# Autodesk Inventor assembly: Structure
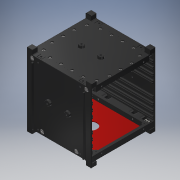
[picture p0: Inventor's stored thumbnail of the model, 180x180]
Saved by Autodesk Inventor 2018 (Build 220112000, 112)
## iProperties
Created: 2018-07-04
Part Number: Structure
Document SubType Name: Assembly
Designer: Bradley
Mass: 378.313 g
Surface Area: 1634.79 cm^2
Volume: 135.905 cm^3
Density: 2.78366 g/cm^3
Author: Bradley
## Documents named in this file (14)
- D:\Users\Bradley\Documents\CougsInSpace\CougSat1-Hardware\CougSat1-Structure\CADModel\Native\Structure.iam
- D:\Users\Bradley\Documents\CougsInSpace\CougSat1-Hardware\CougSat1-Structure\CADModel\Native\Structure_Y.ipt
- D:\Users\Bradley\Documents\CougsInSpace\CougSat1-Hardware\CougSat1-Structure\CADModel\Native\Structure_+Z.ipt
- D:\Users\Bradley\Documents\CougsInSpace\CougSat1-Hardware\CougSat1-Structure\CADModel\Native\Structure_-Z.ipt
- D:\Users\Bradley\Documents\CougsInSpace\CougSat1-Hardware\CougSat1-Structure\CADModel\Native\Structure_+X.ipt
- D:\Users\Bradley\Documents\CougsInSpace\CougSat1-Hardware\CougSat1-Structure\CADModel\Native\Structure_-X.ipt
- D:\Users\Bradley\Documents\CougsInSpace\Resources\ComponentModels\Hardware\Spring_Separation.ipt
- D:\Users\Bradley\Documents\CougsInSpace\Resources\ComponentModels\Electronics\Switch_Micro-L.iam
- D:\Users\Bradley\Documents\CougsInSpace\Resources\ComponentModels\Hardware\Pin_Headed-2x6mm.ipt
- D:\Users\Bradley\Documents\CougsInSpace\Resources\ComponentModels\Fasteners\Bolt_M1.6x0.35_5mm_SH.ipt
- D:\Users\Bradley\Documents\CougsInSpace\Resources\ComponentModels\Fasteners\Bolt_M2x0.4_8mm_SH.ipt
- D:\Users\Bradley\Documents\CougsInSpace\CougSat1-Hardware\CougSat1-Structure\CADModel\Native\Structure_-ZCover.ipt
- D:\Users\Bradley\Documents\CougsInSpace\Resources\ComponentModels\Fasteners\Bolt_M2x0.4_4mm_SH.ipt
- D:\Users\Bradley\Documents\CougsInSpace\Resources\ComponentModels\Fasteners\Bolt_M3x0.35_10mm_LSH.ipt
## Components (47 placed, 13 different names)
1. Structure_+X:1 — Mate:1, Flush:6, Flush:7, Insert:16, Insert:19
2. Structure_Y:1 — Flush:3, Flush:4, Insert:5, Insert:6, Insert:7, Insert:8, Insert:11, Insert:12, Insert:13, Insert:22, Insert:30, Insert:31, Insert:32
3. Structure_+Z:1 — Insert:9, Insert:10, Insert:11, Insert:12, Flush:5, Mate:1, Insert:16, Insert:17, Insert:18, Insert:33, Insert:34, Insert:35, Insert:36, Insert:37, Insert:38, Insert:39, Insert:40, Insert:41, Insert:42, Insert:43, Insert:44, Insert:45, Insert:46, Insert:47, Insert:48, Insert:49, Insert:50
4. Structure_-X:1 — Insert:17, Insert:18, Insert:20
5. Structure_Y:2 — Mate:2, Insert:1, Insert:2, Insert:3, Insert:4, Insert:9, Insert:10, Insert:14, Insert:15, Insert:21, Insert:25, Insert:26, Insert:27
6. Structure_-Z:1 — Insert:13, Insert:14, Insert:15, Insert:19, Insert:20, Insert:51, Insert:52
7. Structure_-ZCover:1 — Insert:51, Insert:52, Insert:53, Insert:54, Insert:55, Insert:56
8. Switch_Micro-L:1 [sub-assembly] — Insert:23, Insert:24, Insert:26, Insert:27, Tangent:1
9. Switch_Micro-L:2 [sub-assembly] — Insert:30, Insert:31
10. Bolt_M1.6x0.35_5mm_SH:1 — Insert:24
11. Bolt_M1.6x0.35_5mm_SH:2 — Insert:23
12. Bolt_M1.6x0.35_5mm_SH:3
13. Bolt_M1.6x0.35_5mm_SH:4
14. Bolt_M2x0.4_4mm_SH:1 — Insert:53
15. Bolt_M2x0.4_4mm_SH:2 — Insert:54
16. Bolt_M2x0.4_4mm_SH:3 — Insert:55
17. Bolt_M2x0.4_4mm_SH:4 — Insert:56
18. Bolt_M2x0.4_8mm_SH:1 — Insert:33
19. Bolt_M2x0.4_8mm_SH:2 — Insert:34
20. Bolt_M2x0.4_8mm_SH:3 — Insert:35
21. Bolt_M2x0.4_8mm_SH:4 — Insert:36
22. Bolt_M2x0.4_8mm_SH:5 — Insert:37
23. Bolt_M2x0.4_8mm_SH:6 — Insert:38
24. Bolt_M2x0.4_8mm_SH:7 — Insert:39
25. Bolt_M2x0.4_8mm_SH:8 — Insert:40
26. Bolt_M2x0.4_8mm_SH:9 — Insert:41
27. Bolt_M2x0.4_8mm_SH:10 — Insert:42
28. Bolt_M2x0.4_8mm_SH:11 — Insert:43
29. Bolt_M2x0.4_8mm_SH:12 — Insert:44
30. Bolt_M2x0.4_8mm_SH:13 — Insert:45
31. Bolt_M2x0.4_8mm_SH:14 — Insert:46
32. Bolt_M2x0.4_8mm_SH:15 — Insert:47
33. Bolt_M2x0.4_8mm_SH:16 — Insert:48
34. Bolt_M2x0.4_8mm_SH:17 — Insert:49
35. Bolt_M2x0.4_8mm_SH:18 — Insert:50
36. Bolt_M3x0.35_10mm_LSH:1 — Insert:1
37. Bolt_M3x0.35_10mm_LSH:2 — Insert:2
38. Bolt_M3x0.35_10mm_LSH:3 — Insert:3
39. Bolt_M3x0.35_10mm_LSH:4 — Insert:4
40. Bolt_M3x0.35_10mm_LSH:5 — Insert:5
41. Bolt_M3x0.35_10mm_LSH:6 — Insert:7
42. Bolt_M3x0.35_10mm_LSH:7 — Insert:6
43. Bolt_M3x0.35_10mm_LSH:8 — Insert:8
44. Pin_Headed-2x6mm:1 — Insert:25, Tangent:1
45. Pin_Headed-2x6mm:2 — Insert:32
46. Spring_Separation:1 — Insert:22
47. Spring_Separation:2 — Insert:21
## Relationships (66: Insert 56, Flush 6, Mate 2, Tangent 2)
- Mate:2: Structure_Y:2
- [Flush]: Structure_Y:2
- Flush:3: Structure_Y:1
- Flush:4: Structure_Y:1
- Insert:1: Structure_Y:2 ↔ Bolt_M3x0.35_10mm_LSH:1
- Insert:2: Structure_Y:2 ↔ Bolt_M3x0.35_10mm_LSH:2
- Insert:3: Structure_Y:2 ↔ Bolt_M3x0.35_10mm_LSH:3
- Insert:4: Structure_Y:2 ↔ Bolt_M3x0.35_10mm_LSH:4
- Insert:5: Structure_Y:1 ↔ Bolt_M3x0.35_10mm_LSH:5
- Insert:6: Structure_Y:1 ↔ Bolt_M3x0.35_10mm_LSH:7
- Insert:7: Structure_Y:1 ↔ Bolt_M3x0.35_10mm_LSH:6
- Insert:8: Structure_Y:1 ↔ Bolt_M3x0.35_10mm_LSH:8
- Insert:9: Structure_+Z:1 ↔ Structure_Y:2
- Insert:10: Structure_+Z:1 ↔ Structure_Y:2
- Insert:11: Structure_Y:1 ↔ Structure_+Z:1
- Insert:12: Structure_Y:1 ↔ Structure_+Z:1
- Flush:5: Structure_+Z:1
- Insert:13: Structure_Y:1 ↔ Structure_-Z:1
- Insert:14: Structure_Y:2 ↔ Structure_-Z:1
- Insert:15: Structure_Y:2 ↔ Structure_-Z:1
- Mate:1: Structure_+X:1 ↔ Structure_+Z:1
- Flush:6: Structure_+X:1
- Flush:7: Structure_+X:1
- Insert:16: Structure_+X:1 ↔ Structure_+Z:1
- Insert:17: Structure_+Z:1 ↔ Structure_-X:1
- Insert:18: Structure_+Z:1 ↔ Structure_-X:1
- Insert:19: Structure_+X:1 ↔ Structure_-Z:1
- Insert:20: Structure_-X:1 ↔ Structure_-Z:1
- Insert:21: Structure_Y:2 ↔ Spring_Separation:2
- Insert:22: Structure_Y:1 ↔ Spring_Separation:1
- Insert:23: Switch_Micro-L:1 ↔ Bolt_M1.6x0.35_5mm_SH:2
- Insert:24: Switch_Micro-L:1 ↔ Bolt_M1.6x0.35_5mm_SH:1
- Insert:25: Structure_Y:2 ↔ Pin_Headed-2x6mm:1
- Insert:26: Structure_Y:2 ↔ Switch_Micro-L:1
- Insert:27: Structure_Y:2 ↔ Switch_Micro-L:1
- Tangent:1: Switch_Micro-L:1 ↔ Pin_Headed-2x6mm:1
- [Insert]: Switch_Micro-L:2 ↔ Bolt_M1.6x0.35_5mm_SH:4
- [Insert]: Switch_Micro-L:2 ↔ Bolt_M1.6x0.35_5mm_SH:3
- [Tangent]: Switch_Micro-L:2 ↔ Pin_Headed-2x6mm:2
- Insert:30: Structure_Y:1 ↔ Switch_Micro-L:2
- Insert:31: Structure_Y:1 ↔ Switch_Micro-L:2
- Insert:32: Structure_Y:1 ↔ Pin_Headed-2x6mm:2
- Insert:33: Structure_+Z:1 ↔ Bolt_M2x0.4_8mm_SH:1
- Insert:34: Structure_+Z:1 ↔ Bolt_M2x0.4_8mm_SH:2
- Insert:35: Structure_+Z:1 ↔ Bolt_M2x0.4_8mm_SH:3
- Insert:36: Structure_+Z:1 ↔ Bolt_M2x0.4_8mm_SH:4
- Insert:37: Structure_+Z:1 ↔ Bolt_M2x0.4_8mm_SH:5
- Insert:38: Structure_+Z:1 ↔ Bolt_M2x0.4_8mm_SH:6
- Insert:39: Structure_+Z:1 ↔ Bolt_M2x0.4_8mm_SH:7
- Insert:40: Structure_+Z:1 ↔ Bolt_M2x0.4_8mm_SH:8
- Insert:41: Structure_+Z:1 ↔ Bolt_M2x0.4_8mm_SH:9
- Insert:42: Structure_+Z:1 ↔ Bolt_M2x0.4_8mm_SH:10
- Insert:43: Structure_+Z:1 ↔ Bolt_M2x0.4_8mm_SH:11
- Insert:44: Structure_+Z:1 ↔ Bolt_M2x0.4_8mm_SH:12
- Insert:45: Structure_+Z:1 ↔ Bolt_M2x0.4_8mm_SH:13
- Insert:46: Structure_+Z:1 ↔ Bolt_M2x0.4_8mm_SH:14
- Insert:47: Structure_+Z:1 ↔ Bolt_M2x0.4_8mm_SH:15
- Insert:48: Structure_+Z:1 ↔ Bolt_M2x0.4_8mm_SH:16
- Insert:49: Structure_+Z:1 ↔ Bolt_M2x0.4_8mm_SH:17
- Insert:50: Structure_+Z:1 ↔ Bolt_M2x0.4_8mm_SH:18
- Insert:51: Structure_-Z:1 ↔ Structure_-ZCover:1
- Insert:52: Structure_-Z:1 ↔ Structure_-ZCover:1
- Insert:53: Structure_-ZCover:1 ↔ Bolt_M2x0.4_4mm_SH:1
- Insert:54: Structure_-ZCover:1 ↔ Bolt_M2x0.4_4mm_SH:2
- Insert:55: Structure_-ZCover:1 ↔ Bolt_M2x0.4_4mm_SH:3
- Insert:56: Structure_-ZCover:1 ↔ Bolt_M2x0.4_4mm_SH:4
## Named parameters: d49_d48 = 0 mm, d50_d39 = 0 mm, d51_d40 = 0 mm
